# Autodesk Inventor assembly: rotator_xw
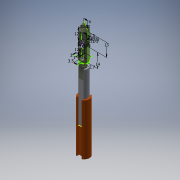
[picture p0: Inventor's stored thumbnail of the model, 180x180]
Saved by Autodesk Inventor 2016 (Build 200138000, 138)
## iProperties
Created: 2015-06-08
Part Number: rotator_xw
Document SubType Name: Assembly
Designer: 121767
Author: 121767
## Documents named in this file (8)
- C:\github\Rotator\Rotator.iam
- C:\github\Rotator\Rotator frame.ipt
- C:\github\Rotator\Gear platform.ipt
- C:\github\Rotator\Suspension axle.ipt
- C:\github\Rotator\Suspension bearing.ipt
- C:\github\Rotator\Slotted center beam.ipt
- C:\github\Rotator\Thick rod.ipt
- C:\Users\121767\Documents\Worm.ipt
## Components (9 placed, 7 different names)
1. Rotator frame:1 — Rigid:7, Rotational:5, Mate:1
2. Gear platform:1 — Rigid:5, Rigid:6
3. Slotted center beam:1 — Rotational:5, Rotational:6
4. Suspension axle:1 — Rotational:3, Rigid:6
5. Suspension axle:2 — Rotational:4, Rigid:5
6. Suspension bearing:1 — Rotational:3
7. Suspension bearing:2 — Rotational:4, Rigid:7
8. thick rod:1 — Rotational:6
9. Worm:1 — Mate:1
## Relationships (8: RevoluteJoint 4, WeldJoint 3, Mate 1)
- Rotational:3 [RevoluteJoint]: Suspension axle:1 ↔ Suspension bearing:1
- Rotational:4 [RevoluteJoint]: Suspension axle:2 ↔ Suspension bearing:2
- Rigid:5 [WeldJoint]: Gear platform:1 ↔ Suspension axle:2
- Rigid:6 [WeldJoint]: Gear platform:1 ↔ Suspension axle:1
- Rigid:7 [WeldJoint]: Rotator frame:1 ↔ Suspension bearing:2
- Rotational:5 [RevoluteJoint] (5 mm): Rotator frame:1 ↔ Slotted center beam:1
- Rotational:6 [RevoluteJoint]: Slotted center beam:1 ↔ thick rod:1
- Mate:1: Rotator frame:1 ↔ Worm:1
